# Autodesk Inventor assembly: Zespół1
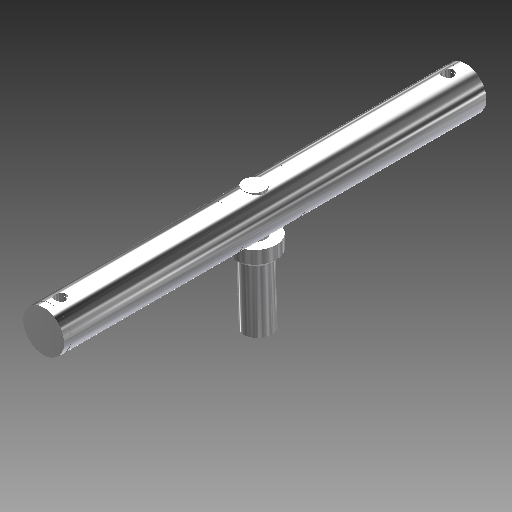
[picture p0: Inventor's stored thumbnail of the model, 512x512]
Saved by Autodesk Inventor 2017 (Build 210142000, 142)
## iProperties
Part Number: Zespół1
Material: Ogólny
Document SubType Name: Assembly
Designer: Dorota
Author: Dorota
## Documents named in this file (6)
- F:\Dropbox\inventor\Rudder-Pedals\palak.iam
- F:\Dropbox\inventor\Rudder-Pedals\czop.ipt
- F:\Dropbox\inventor\Rudder-Pedals\rura.ipt
- F:\Dropbox\inventor\Rudder-Pedals\magne.ipt
- F:\Dropbox\inventor\Rudder-Pedals\srodek.ipt
- F:\Dropbox\inventor\Rudder-Pedals\koncowka-wala.ipt
## Components (7 placed, 5 different names)
1. czop:1 — Zestawiający:8, Zestawiający:9, Zestawiający:10, Styczny:1, Zestawiający:19
2. magne:2 — Zestawiający:8, Zestawiający:9
3. srodek:1 — Zestawiający:10, Styczny:1, Zestawiający:11, Zestawiający:14, Zestawiający:19, Zestawiający:20, Zestawiający:22, Zestawiający:23, Zestawiający:24
4. rura:2 — Zestawiający:11, Zestawiający:14, Zestawiający:16, Zestawiający:18, Zestawiający:20, Zestawiający:21
5. koncowka-wala:1 — Zestawiający:16, Zestawiający:18, Zestawiający:21
6. koncowka-wala:2 — Zestawiający:25, Zestawiający:26
7. rura:3 — Zestawiający:22, Zestawiający:23, Zestawiający:24, Zestawiający:25, Zestawiający:26
## Relationships (16: Mate 15, Tangent 1)
- Zestawiający:8 [Mate]: czop:1 ↔ magne:2
- Zestawiający:9 [Mate]: czop:1 ↔ magne:2
- Zestawiający:10 [Mate]: czop:1 ↔ srodek:1
- Styczny:1 [Tangent]: czop:1 ↔ srodek:1
- Zestawiający:11 [Mate]: srodek:1 ↔ rura:2
- Zestawiający:14 [Mate]: srodek:1 ↔ rura:2
- Zestawiający:16 [Mate]: rura:2 ↔ koncowka-wala:1
- Zestawiający:18 [Mate]: rura:2 ↔ koncowka-wala:1
- Zestawiający:19 [Mate]: czop:1 ↔ srodek:1
- Zestawiający:20 [Mate]: srodek:1 ↔ rura:2
- Zestawiający:21 [Mate]: rura:2 ↔ koncowka-wala:1
- Zestawiający:22 [Mate]: srodek:1 ↔ rura:3
- Zestawiający:23 [Mate]: srodek:1 ↔ rura:3
- Zestawiający:24 [Mate]: srodek:1 ↔ rura:3
- Zestawiający:25 [Mate]: koncowka-wala:2 ↔ rura:3
- Zestawiający:26 [Mate]: koncowka-wala:2 ↔ rura:3
